# Autodesk Inventor assembly: sample complete assembly
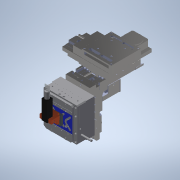
[picture p0: Inventor's stored thumbnail of the model, 180x180]
Saved by Autodesk Inventor 2021 (Build 250183000, 183)
## iProperties
Created: 2019-03-15
Part Number: sample complete assembly
Document SubType Name: Assembly
Designer: Saumya
Author: Saumya
## Documents named in this file (9)
- C:\Users\MicroscopyInnovation\Documents\Inventor\NatProtocolsManuscript\sample_holder_assembly.iam
- C:\Users\MicroscopyInnovation\Documents\Inventor\NatProtocolsManuscript\sample_holder_extension.ipt
- C:\Users\MicroscopyInnovation\Documents\Inventor\NatProtocolsManuscript\sample_holder_bracket.ipt
- C:\Users\MicroscopyInnovation\Documents\Inventor\NatProtocolsManuscript\sample_holder_adapter.ipt
- C:\Users\MicroscopyInnovation\Documents\Inventor\NatProtocolsManuscript\sample_holder_slit_bracket.ipt
- C:\Users\MicroscopyInnovation\Documents\Inventor\NatProtocolsManuscript\sample_holder_glass.ipt
- C:\Users\MicroscopyInnovation\Documents\Inventor\NatProtocolsManuscript\sample_holder_v522.1AA.ipt
- C:\Users\MicroscopyInnovation\Documents\Inventor\NatProtocolsManuscript\sample_holder_sutter_adapter.ipt
- C:\Users\MicroscopyInnovation\Documents\Inventor\NatProtocolsManuscript\sample_holder_mp285.ipt
## Components (8 placed, 8 different names)
1. sample_holder_extension:1 — Cylindrical:1, Mate:18, Flush:1
2. sample_holder_bracket:2 — Mate:11, Mate:12, Mate:13, Flush:1
3. sample_holder_adapter:1 — Mate:5, Mate:6, Mate:10, Mate:11, Mate:12, Mate:13
4. sample_holder_slit_bracket:1 — Cylindrical:1, Mate:15, Mate:16, Mate:17, Mate:18
5. sample_holder_glass:1 — Mate:15, Mate:16, Mate:17
6. sample_holder_v522.1AA:2 — Mate:2, Mate:5, Mate:6, Mate:7, Mate:8, Mate:10
7. sample_holder_sutter_adapter:1 — Mate:2, Mate:4, Mate:7, Mate:8, Mate:9, Angle:1
8. sample_holder_mp285:1 — Mate:4, Mate:9, Angle:1
## Relationships (18: Mate 15, CylindricalJoint 1, Angle 1, Flush 1)
- Cylindrical:1: sample_holder_extension:1 ↔ sample_holder_slit_bracket:1
- Mate:2: sample_holder_v522.1AA:2 ↔ sample_holder_sutter_adapter:1
- Mate:4: sample_holder_sutter_adapter:1 ↔ sample_holder_mp285:1
- Mate:5: sample_holder_adapter:1 ↔ sample_holder_v522.1AA:2
- Mate:6: sample_holder_adapter:1 ↔ sample_holder_v522.1AA:2
- Mate:7: sample_holder_v522.1AA:2 ↔ sample_holder_sutter_adapter:1
- Mate:8: sample_holder_v522.1AA:2 ↔ sample_holder_sutter_adapter:1
- Mate:9: sample_holder_sutter_adapter:1 ↔ sample_holder_mp285:1
- Mate:10: sample_holder_adapter:1 ↔ sample_holder_v522.1AA:2
- Mate:11: sample_holder_bracket:2 ↔ sample_holder_adapter:1
- Mate:12: sample_holder_bracket:2 ↔ sample_holder_adapter:1
- Mate:13: sample_holder_bracket:2 ↔ sample_holder_adapter:1
- Angle:1 (0 deg): sample_holder_sutter_adapter:1 ↔ sample_holder_mp285:1
- Mate:15: sample_holder_slit_bracket:1 ↔ sample_holder_glass:1
- Mate:16: sample_holder_slit_bracket:1 ↔ sample_holder_glass:1
- Mate:17 (-5 mm): sample_holder_slit_bracket:1 ↔ sample_holder_glass:1
- Mate:18: sample_holder_extension:1 ↔ sample_holder_slit_bracket:1
- Flush:1: sample_holder_extension:1 ↔ sample_holder_bracket:2
